# Autodesk Inventor assembly: A2017_T2_14
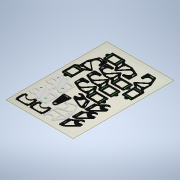
[picture p0: Inventor's stored thumbnail of the model, 180x180]
Saved by Autodesk Inventor 2020 (Build 240168000, 168)
## iProperties
Created: 2021-08-27
Part Number: A2017_T2_14
Document SubType Name: Assembly
Designer: Masato
Author: Masato
## Documents named in this file (8)
- D:\GitHub\inventor\SUSTAINA-OP\Cam\A2017_T2_14.iam
- D:\GitHub\inventor\SUSTAINA-OP\Cam\DisposableBoard.ipt
- D:\GitHub\inventor\SUSTAINA-OP\LowerBody\Ankle\Ankle_back_frame.ipt
- D:\GitHub\inventor\SUSTAINA-OP\LowerBody\Foot\Foot_front_frame.ipt
- D:\GitHub\inventor\SUSTAINA-OP\LowerBody\Knee\Knee_side_frame.ipt
- D:\GitHub\inventor\SUSTAINA-OP\LowerBody\Leg_joint\Leg_joint_pitch_frame.ipt
- D:\GitHub\inventor\SUSTAINA-OP\UpperBody\Arm\Shoulder_side_frame.ipt
- D:\GitHub\inventor\SUSTAINA-OP\LowerBody\Ankle\Ankle_side_frame.ipt
## Components (19 placed, 7 different names)
1. DisposableBoard:1 — メイト:2, メイト:1, フラッシュ:1, フラッシュ:2, メイト:4, メイト:5, メイト:6, メイト:7, メイト:9, メイト:10, メイト:11, メイト:18, メイト:19, メイト:20, メイト:21, メイト:22, メイト:24, メイト:25, メイト:27, メイト:28, メイト:30, メイト:35
2. Foot_front_frame:1 — メイト:15, メイト:19, 正接:3, メイト:29
3. Knee_side_frame:1 — メイト:7, メイト:17, メイト:18, 正接:3, 正接:4, 正接:9
4. Ankle_side_frame:1 — メイト:24, メイト:25, メイト:26, メイト:31, メイト:33
5. Shoulder_side_frame:4 — メイト:22, メイト:23, 正接:8, メイト:29, 正接:9
6. Ankle_side_frame:7 — メイト:28, メイト:33, 正接:10, メイト:36
7. Ankle_side_frame:10 — メイト:30, メイト:31, メイト:32, 正接:10, メイト:34, 正接:11
8. Ankle_side_frame:11 — メイト:34, メイト:35, 正接:11, メイト:36
9. Ankle_back_frame:1 — メイト:4, メイト:5, メイト:6, 正接:2
10. Ankle_back_frame:2 — メイト:13, メイト:17
11. Leg_joint_pitch_frame:1 — メイト:9, メイト:10, メイト:12, 正接:2
12. Leg_joint_pitch_frame:2 — メイト:11, メイト:12, メイト:13, メイト:15
13. Leg_joint_pitch_frame:3 — メイト:26
14. Leg_joint_pitch_frame:4
15. Shoulder_side_frame:1 — メイト:20, メイト:21, 正接:4
16. Shoulder_side_frame:2
17. Shoulder_side_frame:3 — メイト:23, 正接:7
18. Ankle_side_frame:2 — メイト:27, 正接:7, 正接:8, 角度:1
19. Ankle_side_frame:9 — メイト:32
## Component patterns: (2 elements, first: Ankle_back_frame:1), (2 elements, first: Leg_joint_pitch_frame:1 + Leg_joint_pitch_frame:2), (3 elements, first: Shoulder_side_frame:1), (2 elements, first: Ankle_side_frame:2)
## Relationships (43: Mate 32, Tangent 8, Flush 2, Angle 1)
- メイト:2 [Mate]: DisposableBoard:1
- メイト:1 [Mate]: DisposableBoard:1
- フラッシュ:1 [Flush]: DisposableBoard:1
- フラッシュ:2 [Flush]: DisposableBoard:1
- メイト:4 [Mate]: DisposableBoard:1 ↔ Ankle_back_frame:1
- メイト:5 [Mate] (2 mm): DisposableBoard:1 ↔ Ankle_back_frame:1
- メイト:6 [Mate] (2 mm): DisposableBoard:1 ↔ Ankle_back_frame:1
- メイト:7 [Mate]: DisposableBoard:1 ↔ Knee_side_frame:1
- メイト:9 [Mate]: DisposableBoard:1 ↔ Leg_joint_pitch_frame:1
- メイト:10 [Mate] (2 mm): DisposableBoard:1 ↔ Leg_joint_pitch_frame:1
- メイト:11 [Mate]: DisposableBoard:1 ↔ Leg_joint_pitch_frame:2
- メイト:12 [Mate] (2.5 mm): Leg_joint_pitch_frame:1 ↔ Leg_joint_pitch_frame:2
- 正接:2 [Tangent] (2.5 mm): Ankle_back_frame:1 ↔ Leg_joint_pitch_frame:1
- メイト:13 [Mate] (2.5 mm): Ankle_back_frame:2 ↔ Leg_joint_pitch_frame:2
- メイト:15 [Mate] (2.5 mm): Foot_front_frame:1 ↔ Leg_joint_pitch_frame:2
- メイト:17 [Mate] (2.5 mm): Knee_side_frame:1 ↔ Ankle_back_frame:2
- メイト:18 [Mate] (2.5 mm): DisposableBoard:1 ↔ Knee_side_frame:1
- メイト:19 [Mate]: DisposableBoard:1 ↔ Foot_front_frame:1
- 正接:3 [Tangent] (2.5 mm): Foot_front_frame:1 ↔ Knee_side_frame:1
- メイト:20 [Mate]: DisposableBoard:1 ↔ Shoulder_side_frame:1
- メイト:21 [Mate] (2 mm): DisposableBoard:1 ↔ Shoulder_side_frame:1
- 正接:4 [Tangent] (2.5 mm): Knee_side_frame:1 ↔ Shoulder_side_frame:1
- メイト:22 [Mate]: DisposableBoard:1 ↔ Shoulder_side_frame:4
- メイト:23 [Mate] (2.5 mm): Shoulder_side_frame:4 ↔ Shoulder_side_frame:3
- メイト:24 [Mate]: DisposableBoard:1 ↔ Ankle_side_frame:1
- メイト:25 [Mate] (2.5 mm): DisposableBoard:1 ↔ Ankle_side_frame:1
- メイト:26 [Mate] (2.5 mm): Ankle_side_frame:1 ↔ Leg_joint_pitch_frame:3
- メイト:27 [Mate]: DisposableBoard:1 ↔ Ankle_side_frame:2
- 正接:7 [Tangent] (2.5 mm): Shoulder_side_frame:3 ↔ Ankle_side_frame:2
- 正接:8 [Tangent] (2.5 mm): Shoulder_side_frame:4 ↔ Ankle_side_frame:2
- 角度:1 [Angle] (-90 deg): Ankle_side_frame:2
- メイト:28 [Mate]: DisposableBoard:1 ↔ Ankle_side_frame:7
- メイト:29 [Mate] (2.5 mm): Foot_front_frame:1 ↔ Shoulder_side_frame:4
- 正接:9 [Tangent] (2.5 mm): Knee_side_frame:1 ↔ Shoulder_side_frame:4
- メイト:30 [Mate]: DisposableBoard:1 ↔ Ankle_side_frame:10
- メイト:31 [Mate] (2.5 mm): Ankle_side_frame:1 ↔ Ankle_side_frame:10
- メイト:32 [Mate] (2.5 mm): Ankle_side_frame:10 ↔ Ankle_side_frame:9
- メイト:33 [Mate] (2.5 mm): Ankle_side_frame:1 ↔ Ankle_side_frame:7
- 正接:10 [Tangent] (2.5 mm): Ankle_side_frame:7 ↔ Ankle_side_frame:10
- メイト:34 [Mate] (2.5 mm): Ankle_side_frame:10 ↔ Ankle_side_frame:11
- メイト:35 [Mate]: DisposableBoard:1 ↔ Ankle_side_frame:11
- 正接:11 [Tangent] (2.5 mm): Ankle_side_frame:10 ↔ Ankle_side_frame:11
- メイト:36 [Mate] (13.084 mm): Ankle_side_frame:7 ↔ Ankle_side_frame:11
